# Autodesk Inventor assembly: ROV Control Pipe Assembly
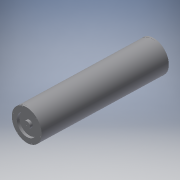
[picture p0: Inventor's stored thumbnail of the model, 180x180]
Saved by Autodesk Inventor 2016 (Build 200138000, 138)
## iProperties
Created: 2017-01-19
Part Number: ROV Control Pipe Assembly
Document SubType Name: Assembly
Designer: Student
Author: Student
## Documents named in this file (6)
- C:\Users\Student\Desktop\ROV Control Pipe Assembly.iam
- C:\Users\Student\Desktop\Noah Code\4 inch PVC pipe.ipt
- C:\Users\Student\Desktop\LED Driver.ipt
- C:\Users\Student\Documents\Raspberry Pi.ipt
- C:\Users\Student\Documents\arduino uno.ipt
- C:\Users\Student\Desktop\O ring Plug 1.ipt
## Components (6 placed, 5 different names)
1. 4 inch PVC pipe:1 — Mate:1, Mate:2
2. LED Driver:1
3. Raspberry Pi:1
4. arduino uno:1
5. O ring Plug 1:1 — Mate:1
6. O ring Plug 1:2 — Mate:2
## Relationships (2: Mate 2)
- Mate:1: 4 inch PVC pipe:1 ↔ O ring Plug 1:1
- Mate:2: 4 inch PVC pipe:1 ↔ O ring Plug 1:2
